# Autodesk Inventor assembly: Assembly
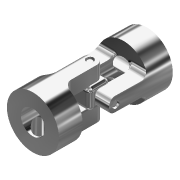
[picture p0: Inventor's stored thumbnail of the model, 180x180]
Saved by Autodesk Inventor 2020 (Build 240168000, 168)
## iProperties
Created: 2021-06-28
Part Number: Assembly
Document SubType Name: Assembly
Designer: Coy
Author: Coy
## Documents named in this file (3)
- E:\Documents\3D Files\Project 3D Models\Industrial 6 Axis Robot Arm\4th 5th amd 6th axis model\5x24mm Universal Joint\Assembly.iam
- E:\Documents\3D Files\Project 3D Models\Industrial 6 Axis Robot Arm\4th 5th amd 6th axis model\5x24mm Universal Joint\Yoke.ipt
- E:\Documents\3D Files\Project 3D Models\Industrial 6 Axis Robot Arm\4th 5th amd 6th axis model\5x24mm Universal Joint\Ball.ipt
## Components (3 placed, 2 different names)
1. Yoke:1 — Mate:1, Mate:2
2. Yoke:2 — Mate:3, Mate:4
3. Ball:1 — Mate:1, Mate:2, Mate:3, Mate:4
## Relationships (4: Mate 4)
- Mate:1: Yoke:1 ↔ Ball:1
- Mate:2: Yoke:1 ↔ Ball:1
- Mate:3: Yoke:2 ↔ Ball:1
- Mate:4: Yoke:2 ↔ Ball:1
